# Autodesk Inventor assembly: Assembly2
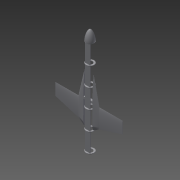
[picture p0: Inventor's stored thumbnail of the model, 180x180]
Saved by Autodesk Inventor 2014 SP1 (Build 180222100, 222)
## iProperties
Created: 2018-05-14
Part Number: Assembly2
Document SubType Name: Assembly
Designer: Dadang
Author: Dadang
## Documents named in this file (6)
- D:\Gambar Inventor\Wahana Roket\roket kontruction\Assembly2.iam
- D:\Gambar Inventor\Wahana Roket\roket kontruction\Part1.ipt
- D:\Gambar Inventor\Wahana Roket\roket kontruction\Part2.ipt
- D:\Gambar Inventor\Wahana Roket\roket kontruction\moncong.ipt
- D:\Gambar Inventor\Wahana Roket\roket kontruction\wing.ipt
- D:\Gambar Inventor\Wahana Roket\roket kontruction\wing2.ipt
## Components (10 placed, 5 different names)
1. Part2:1 — Mate:1, Mate:2, Mate:3, Mate:6, Mate:7, Mate:8, Mate:10
2. moncong:1 — Mate:4, Mate:5
3. wing:1 — Mate:6, Mate:7, Mate:8, Mate:9
4. wing2:1 — Mate:9, Mate:10
5. Part1:1 — Mate:1, Mate:2, Mate:3, Mate:4, Mate:5
6. Part1:2
7. Part1:3
8. Part1:4
9. Part1:5
10. Part1:6
## Component patterns: (6 elements, first: Part1:1)
## Relationships (10: Mate 10)
- Mate:1: Part2:1 ↔ Part1:1
- Mate:2: Part2:1 ↔ Part1:1
- Mate:3: Part2:1 ↔ Part1:1
- Mate:4: moncong:1 ↔ Part1:1
- Mate:5: moncong:1 ↔ Part1:1
- Mate:6: Part2:1 ↔ wing:1
- Mate:7: Part2:1 ↔ wing:1
- Mate:8: Part2:1 ↔ wing:1
- Mate:9: wing:1 ↔ wing2:1
- Mate:10: Part2:1 ↔ wing2:1
